# Autodesk Inventor assembly: 100-01
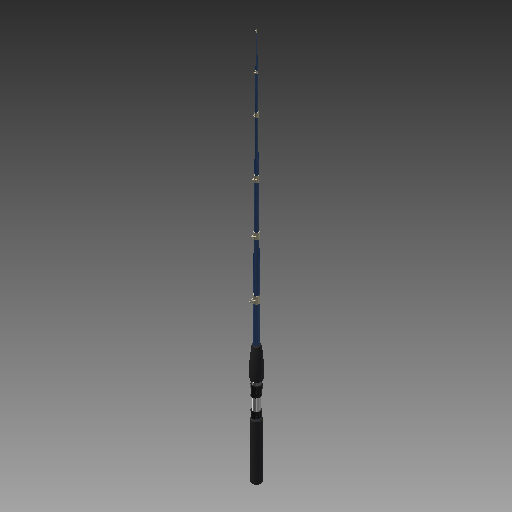
[picture p0: Inventor's stored thumbnail of the model, 512x512]
Saved by Autodesk Inventor 2019 (Build 230136000, 136)
## iProperties
Company: Autodesk Inc.
Created: 2017-06-27
Part Number: 100-01
Document SubType Name: Assembly
Designer: Autodesk Inc.
Mass: 100.231 g
Surface Area: 2013.31 cm^2
Volume: 800.942 cm^3
Density: 0.125141 g/cm^3
Author: Inventor
## Documents named in this file (5)
- C:\TEMP\Fishing Rod\Workspaces\Rod Assembly.iam
- C:\TEMP\Fishing Rod\Workspaces\Fishing Rod.ipt
- C:\TEMP\Fishing Rod\Workspaces\Base Clip.ipt
- C:\TEMP\Fishing Rod\Workspaces\Top Clip Holder.ipt
- C:\TEMP\Fishing Rod\Workspaces\Top Clip.ipt
## Components (4 placed, 4 different names)
1. Fishing Rod:1 — Mate:1, Mate:2, Flush:10, Flush:1, Flush:11, Mate:6
2. Base Clip:1 — Mate:1, Mate:2, Mate:3, Mate:7
3. Top Clip Holder:1 — Insert:1, Mate:6
4. Top Clip:1 — Mate:3, Insert:1, Flush:9
## Relationships (10: Mate 5, Flush 4, Insert 1)
- Mate:1: Fishing Rod:1 ↔ Base Clip:1
- Mate:2 (2 mm): Fishing Rod:1 ↔ Base Clip:1
- Mate:3: Base Clip:1 ↔ Top Clip:1
- Insert:1: Top Clip Holder:1 ↔ Top Clip:1
- Flush:10: Fishing Rod:1
- Flush:1: Fishing Rod:1
- Flush:11: Fishing Rod:1
- Mate:6 (10 mm): Fishing Rod:1 ↔ Top Clip Holder:1
- Mate:7: Base Clip:1
- Flush:9: Top Clip:1
